# Autodesk Inventor assembly: Mains Inlet Foot
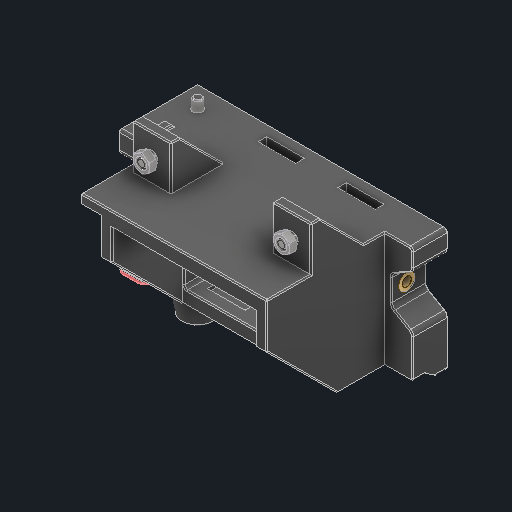
[picture p0: Inventor's stored thumbnail of the model, 512x512]
Saved by Autodesk Inventor 2025.1 (Build 291241020, 241B)
## iProperties
Created: 2025-05-09
Part Number: Mains Inlet Foot
Document SubType Name: Assembly
Designer: AdminForWorker
Title: Mains Inlet Foot
Author: AdminForWorker
## Documents named in this file (9)
- C:\Users\Joshua Eah\Documents\Voron 0.2\CAD\Master Assembly\Mains Inlet Foot.iam
- C:\Users\Joshua Eah\Documents\Voron 0.2\CAD\Master Assembly\Mains Inlet.ipt
- C:\Users\Joshua Eah\Documents\Voron 0.2\CAD\Master Assembly\Printed Parts (6).iam
- C:\Users\Joshua Eah\Documents\Voron 0.2\CAD\Master Assembly\Hardware\Threaded Insert Assemblies\Threaded Inserts (2).iam
- C:\Users\Joshua Eah\Documents\Voron 0.2\CAD\Master Assembly\Rubber Foot.ipt
- C:\Users\Joshua Eah\Documents\Voron 0.2\CAD\Master Assembly\Hardware\M2x10 Self Tapper.ipt
- C:\Users\Joshua Eah\Documents\Voron 0.2\CAD\Master Assembly\Hardware\M3x10 BHCS.ipt
- C:\Users\Joshua Eah\Documents\Voron 0.2\CAD\Master Assembly\Hardware\M3x40 BHCS.ipt
- C:\Users\Joshua Eah\Documents\Voron 0.2\CAD\Master Assembly\Hardware\M3 Hexnut.ipt
## Components (12 placed, 8 different names)
1. Mains Inlet:1
2. Printed Parts (6):1 [sub-assembly] — Insert:1, Insert:2
3. Threaded Inserts (2):1 [sub-assembly]
4. Rubber Foot:2
5. M2x10 Self Tapper:1 — Insert:1
6. M2x10 Self Tapper:2 — Insert:2
7. M3x10 BHCS:1
8. M3x10 BHCS:2
9. M3x10 BHCS:3
10. M3x40 BHCS:1
11. M3 Hexnut:1
12. M3 Hexnut:2
## Relationships (2: Insert 2)
- Insert:1: Printed Parts (6):1 ↔ M2x10 Self Tapper:1
- Insert:2: Printed Parts (6):1 ↔ M2x10 Self Tapper:2
